# Autodesk Inventor assembly: jersey_wheels_assembly
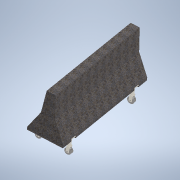
[picture p0: Inventor's stored thumbnail of the model, 180x180]
Saved by Autodesk Inventor 2022 (Build 260153000, 153)
## iProperties
Created: 2021-11-07
Part Number: jersey_wheels_assembly
Document SubType Name: Assembly
Designer: kibandi
Author: kibandi
## Documents named in this file (4)
- C:\academics\YEAR 4\4.2\DOMS II\DOMS II projects\mechanical design\jersey_wheels_assembly.iam
- C:\academics\YEAR 4\4.2\DOMS II\DOMS II projects\mechanical design\Jersey Curb.ipt
- C:\academics\YEAR 4\4.2\DOMS II\DOMS II projects\mechanical design\Rail_wheel_assembly.iam
- C:\academics\YEAR 4\4.2\DOMS II\DOMS II projects\mechanical design\barrier_pneumatic_connector.ipt
## Components (6 placed, 3 different names)
1. Jersey Curb:1 — Mate:1, Mate:2, Mate:3, Mate:4, Mate:5, Mate:6, Mate:7, Mate:8, Mate:9, Mate:10, Mate:11
2. Rail_wheel_assembly:1 [sub-assembly] — Mate:1, Mate:2, Mate:7
3. Rail_wheel_assembly:2 [sub-assembly] — Mate:3, Mate:4
4. Rail_wheel_assembly:3 [sub-assembly] — Mate:5, Mate:6
5. Rail_wheel_assembly:4 [sub-assembly] — Mate:8, Mate:9
6. barrier_pneumatic_connector:1 — Mate:10, Mate:11
## Relationships (11: Mate 11)
- Mate:1: Jersey Curb:1 ↔ Rail_wheel_assembly:1
- Mate:2: Jersey Curb:1 ↔ Rail_wheel_assembly:1
- Mate:3: Jersey Curb:1 ↔ Rail_wheel_assembly:2
- Mate:4: Jersey Curb:1 ↔ Rail_wheel_assembly:2
- Mate:5: Jersey Curb:1 ↔ Rail_wheel_assembly:3
- Mate:6: Jersey Curb:1 ↔ Rail_wheel_assembly:3
- Mate:7: Jersey Curb:1 ↔ Rail_wheel_assembly:1
- Mate:8: Jersey Curb:1 ↔ Rail_wheel_assembly:4
- Mate:9: Jersey Curb:1 ↔ Rail_wheel_assembly:4
- Mate:10: Jersey Curb:1 ↔ barrier_pneumatic_connector:1
- Mate:11: Jersey Curb:1 ↔ barrier_pneumatic_connector:1
